# Autodesk Inventor assembly: assembly
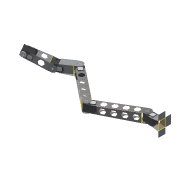
[picture p0: Inventor's stored thumbnail of the model, 180x180]
Saved by Autodesk Inventor 2018 (Build 220112000, 112)
## iProperties
Created: 2018-10-15
Part Number: assembly
Document SubType Name: Assembly
Designer: Bardo91
Author: Bardo91
## Documents named in this file (6)
- E:\programming\servarm\hardware\assembly.iam
- E:\programming\servarm\hardware\XYZ Servo.ipt
- E:\programming\servarm\hardware\arm1.ipt
- E:\programming\servarm\hardware\arm2.ipt
- E:\programming\servarm\hardware\arm3.ipt
- E:\programming\servarm\hardware\attachment.ipt
## Components (10 placed, 5 different names)
1. XYZ Servo:1 — Mate:2, Mate:3, Mate:4, Mate:7, Mate:16
2. arm1:1 — Mate:7, Mate:8, Mate:9, Mate:16, Mate:17
3. arm1:2 — Mate:2, Mate:3, Mate:4, Mate:5, Mate:6
4. XYZ Servo:2 — Mate:5, Mate:6, Mate:22, Mate:23, Mate:24
5. XYZ Servo:3 — Mate:14, Mate:15, Mate:21
6. XYZ Servo:4 — Mate:11, Mate:12, Mate:13, Mate:19, Mate:20
7. XYZ Servo:5 — Mate:8, Mate:9, Mate:10, Mate:17, Mate:18
8. arm2:1 — Mate:10, Mate:11, Mate:12, Mate:18, Mate:19
9. arm3:1 — Mate:13, Mate:14, Mate:15, Mate:20, Mate:21
10. attachment:1 — Mate:22, Mate:23, Mate:24
## Relationships (23: Mate 23)
- Mate:2: XYZ Servo:1 ↔ arm1:2
- Mate:3: XYZ Servo:1 ↔ arm1:2
- Mate:4: XYZ Servo:1 ↔ arm1:2
- Mate:5: arm1:2 ↔ XYZ Servo:2
- Mate:6: arm1:2 ↔ XYZ Servo:2
- Mate:7: XYZ Servo:1 ↔ arm1:1
- Mate:8: arm1:1 ↔ XYZ Servo:5
- Mate:9: arm1:1 ↔ XYZ Servo:5
- Mate:10: XYZ Servo:5 ↔ arm2:1
- Mate:11: XYZ Servo:4 ↔ arm2:1
- Mate:12: XYZ Servo:4 ↔ arm2:1
- Mate:13: XYZ Servo:4 ↔ arm3:1
- Mate:14: XYZ Servo:3 ↔ arm3:1
- Mate:15: XYZ Servo:3 ↔ arm3:1
- Mate:16: XYZ Servo:1 ↔ arm1:1
- Mate:17: arm1:1 ↔ XYZ Servo:5
- Mate:18: XYZ Servo:5 ↔ arm2:1
- Mate:19: XYZ Servo:4 ↔ arm2:1
- Mate:20: XYZ Servo:4 ↔ arm3:1
- Mate:21: XYZ Servo:3 ↔ arm3:1
- Mate:22: XYZ Servo:2 ↔ attachment:1
- Mate:23: XYZ Servo:2 ↔ attachment:1
- Mate:24: XYZ Servo:2 ↔ attachment:1
